# Autodesk Inventor assembly: Assembly3
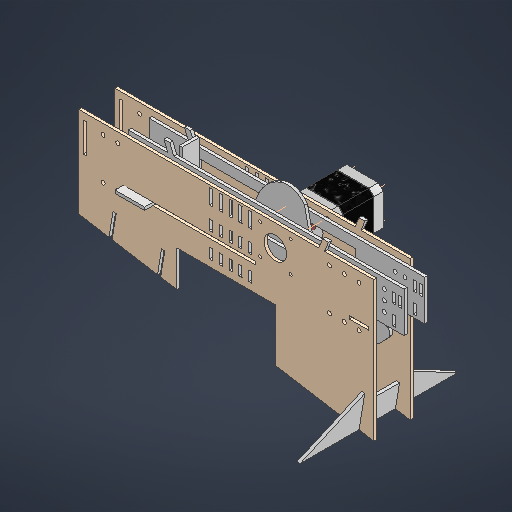
[picture p0: Inventor's stored thumbnail of the model, 512x512]
Saved by Autodesk Inventor 2027 (Build 310192000, 192)
## iProperties
Created: 2026-05-11
Part Number: Assembly3
Document SubType Name: Assembly
Designer: alexy
Author: alexy
## Documents named in this file (8)
- C:\Users\alexy\OneDrive\文件\Carinventor\1stmodel\Assembly3-2.iam
- C:\Users\alexy\OneDrive\文件\Carinventor\1stmodel\Sideboard3.ipt
- C:\Users\alexy\OneDrive\文件\Carinventor\1stmodel\Nema 17 stepper motor.ipt
- C:\Users\alexy\OneDrive\文件\Carinventor\1stmodel\Moving_rail3.ipt
- C:\Users\alexy\OneDrive\文件\Carinventor\1stmodel\Middle_bar3.ipt
- C:\Users\alexy\OneDrive\文件\Carinventor\1stmodel\contact_board3.ipt
- C:\Users\alexy\OneDrive\文件\Carinventor\1stmodel\cam3-2.ipt
- C:\Users\alexy\OneDrive\文件\Carinventor\1stmodel\Support_base.ipt
## Components (9 placed, 7 different names)
1. Sideboard3:1 — Mate:1, Insert:1, Angle:1, Mate:2, Mate:10, Mate:33, Mate:35, Mate:37
2. Nema 17 stepper motor:1 — Mate:1, Insert:1, Angle:1, Insert:2
3. Moving_rail3:1 — Mate:2, Mate:4, Mate:5, Mate:6, Mate:17
4. Middle_bar3:1 — Mate:4, Mate:5, Mate:6, Mate:10, Mate:11, Mate:12, Mate:13, Flush:1, Flush:2
5. contact_board3:2 — Mate:11, Mate:12, Mate:13
6. Middle_bar3:2 — Flush:1, Flush:2, Mate:17
7. cam3-2:1 — Insert:2
8. Support_base:1 — Mate:33, Mate:34, Mate:35, Mate:36, Mate:37, Mate:38
9. Sideboard3:3 — Mate:34, Mate:36, Mate:38
## Relationships (21: Mate 16, Insert 2, Flush 2, Angle 1)
- Mate:1: Sideboard3:1 ↔ Nema 17 stepper motor:1
- Insert:1: Sideboard3:1 ↔ Nema 17 stepper motor:1
- Angle:1 (180 deg): Sideboard3:1 ↔ Nema 17 stepper motor:1
- Mate:2: Sideboard3:1 ↔ Moving_rail3:1
- Mate:4: Moving_rail3:1 ↔ Middle_bar3:1
- Mate:5: Moving_rail3:1 ↔ Middle_bar3:1
- Mate:6: Moving_rail3:1 ↔ Middle_bar3:1
- Mate:10 (3 mm): Sideboard3:1 ↔ Middle_bar3:1
- Mate:11: Middle_bar3:1 ↔ contact_board3:2
- Mate:12: Middle_bar3:1 ↔ contact_board3:2
- Mate:13: Middle_bar3:1 ↔ contact_board3:2
- Flush:1: Middle_bar3:1 ↔ Middle_bar3:2
- Flush:2: Middle_bar3:1 ↔ Middle_bar3:2
- Mate:17: Moving_rail3:1 ↔ Middle_bar3:2
- Insert:2 (10 mm): Nema 17 stepper motor:1 ↔ cam3-2:1
- Mate:33: Sideboard3:1 ↔ Support_base:1
- Mate:34: Support_base:1 ↔ Sideboard3:3
- Mate:35: Sideboard3:1 ↔ Support_base:1
- Mate:36: Support_base:1 ↔ Sideboard3:3
- Mate:37: Sideboard3:1 ↔ Support_base:1
- Mate:38: Support_base:1 ↔ Sideboard3:3
